# Autodesk Inventor assembly: 2x8
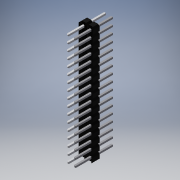
[picture p0: Inventor's stored thumbnail of the model, 180x180]
Saved by Autodesk Inventor 2019 (Build 230136000, 136)
## iProperties
Created: 2019-06-02
Part Number: 2x8
Document SubType Name: Assembly
Designer: jg_ma
Author: jg_ma
## Documents named in this file (2)
- D:\Desktop\Eletronica_Mecanica\MainBoard_V1.1\Pinos\2x17.iam
- D:\Desktop\Eletronica_Mecanica\MainBoard_V1.1\Pinos\Pino_180(2).ipt
## Components (17 placed, 1 different names)
1. Pino_180(2):1 — Mate:1, Flush:7, Flush:15, Mate:15, Flush:31, Flush:32
2. Pino_180(2):2 — Mate:1, Mate:2, Flush:6, Flush:7, Flush:14, Flush:15
3. Pino_180(2):3 — Mate:2, Mate:3, Flush:5, Flush:6, Flush:13, Flush:14
4. Pino_180(2):4 — Mate:3, Mate:4, Flush:4, Flush:5, Flush:12, Flush:13
5. Pino_180(2):5 — Mate:7, Flush:1, Flush:9
6. Pino_180(2):6 — Mate:6, Mate:7, Flush:1, Flush:2, Flush:9, Flush:10
7. Pino_180(2):7 — Mate:5, Mate:6, Flush:2, Flush:3, Flush:8, Flush:10, Flush:11
8. Pino_180(2):8 — Mate:4, Mate:5, Flush:3, Flush:4, Flush:8, Flush:11, Flush:12
9. Pino_180(2):9 — Mate:16, Flush:33, Flush:34
10. Pino_180(2):10
11. Pino_180(2):11
12. Pino_180(2):12
13. Pino_180(2):13 — Mate:15, Flush:31, Flush:32
14. Pino_180(2):14
15. Pino_180(2):15
16. Pino_180(2):16
17. Pino_180(2):17 — Mate:16, Flush:33, Flush:34
## Relationships (50: Flush 34, Mate 16)
- Mate:1: Pino_180(2):1 ↔ Pino_180(2):2
- Mate:2: Pino_180(2):2 ↔ Pino_180(2):3
- Mate:3: Pino_180(2):3 ↔ Pino_180(2):4
- Mate:4: Pino_180(2):4 ↔ Pino_180(2):8
- Mate:5: Pino_180(2):7 ↔ Pino_180(2):8
- Mate:6: Pino_180(2):6 ↔ Pino_180(2):7
- Mate:7: Pino_180(2):5 ↔ Pino_180(2):6
- Flush:1: Pino_180(2):5 ↔ Pino_180(2):6
- Flush:2: Pino_180(2):6 ↔ Pino_180(2):7
- Flush:3: Pino_180(2):7 ↔ Pino_180(2):8
- Flush:4: Pino_180(2):4 ↔ Pino_180(2):8
- Flush:5: Pino_180(2):3 ↔ Pino_180(2):4
- Flush:6: Pino_180(2):2 ↔ Pino_180(2):3
- Flush:7: Pino_180(2):1 ↔ Pino_180(2):2
- Flush:8: Pino_180(2):7 ↔ Pino_180(2):8
- Flush:9: Pino_180(2):5 ↔ Pino_180(2):6
- Flush:10: Pino_180(2):6 ↔ Pino_180(2):7
- Flush:11: Pino_180(2):7 ↔ Pino_180(2):8
- Flush:12: Pino_180(2):4 ↔ Pino_180(2):8
- Flush:13: Pino_180(2):3 ↔ Pino_180(2):4
- Flush:14: Pino_180(2):2 ↔ Pino_180(2):3
- Flush:15: Pino_180(2):1 ↔ Pino_180(2):2
- [Mate]: Pino_180(2):9 ↔ Pino_180(2):10
- [Mate]: Pino_180(2):10 ↔ Pino_180(2):11
- [Mate]: Pino_180(2):11 ↔ Pino_180(2):12
- [Mate]: Pino_180(2):12 ↔ Pino_180(2):16
- [Mate]: Pino_180(2):15 ↔ Pino_180(2):16
- [Mate]: Pino_180(2):14 ↔ Pino_180(2):15
- [Mate]: Pino_180(2):13 ↔ Pino_180(2):14
- [Flush]: Pino_180(2):13 ↔ Pino_180(2):14
- [Flush]: Pino_180(2):14 ↔ Pino_180(2):15
- [Flush]: Pino_180(2):15 ↔ Pino_180(2):16
- [Flush]: Pino_180(2):12 ↔ Pino_180(2):16
- [Flush]: Pino_180(2):11 ↔ Pino_180(2):12
- [Flush]: Pino_180(2):10 ↔ Pino_180(2):11
- [Flush]: Pino_180(2):9 ↔ Pino_180(2):10
- [Flush]: Pino_180(2):15 ↔ Pino_180(2):16
- [Flush]: Pino_180(2):13 ↔ Pino_180(2):14
- [Flush]: Pino_180(2):14 ↔ Pino_180(2):15
- [Flush]: Pino_180(2):15 ↔ Pino_180(2):16
- [Flush]: Pino_180(2):12 ↔ Pino_180(2):16
- [Flush]: Pino_180(2):11 ↔ Pino_180(2):12
- [Flush]: Pino_180(2):10 ↔ Pino_180(2):11
- [Flush]: Pino_180(2):9 ↔ Pino_180(2):10
- Mate:15: Pino_180(2):1 ↔ Pino_180(2):13
- Flush:31: Pino_180(2):1 ↔ Pino_180(2):13
- Flush:32: Pino_180(2):1 ↔ Pino_180(2):13
- Mate:16: Pino_180(2):9 ↔ Pino_180(2):17
- Flush:33: Pino_180(2):9 ↔ Pino_180(2):17
- Flush:34: Pino_180(2):9 ↔ Pino_180(2):17
## Named parameters: d22_d6 = 0 mm, d23_d7 = 0 mm, d24_d8 = 0 mm, d25_d9 = 0 mm, d26_d10 = 0 mm, d27_d11 = 0 mm, d28_d12 = 0 mm, d29_d13 = 0 mm, d30_d14 = 0 mm, d31_d15 = 0 mm, d32_d16 = 0 mm, d33_d17 = 0 mm, d34_d18 = 0 mm, d35_d19 = 0 mm, d36_d20 = 0 mm, d37_d21 = 0 mm, d38_d0 = 0 mm, d39_d1 = 0 mm, d40_d2 = 0 mm, d41_d3 = 0 mm, d42_d4 = 0 mm, d43_d5 = 0 mm
